# Autodesk Inventor assembly: ORBD Assembly
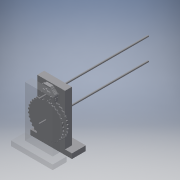
[picture p0: Inventor's stored thumbnail of the model, 180x180]
Saved by Autodesk Inventor 2017 (Build 210142000, 142)
## iProperties
Created: 2018-03-04
Part Number: ORBD Assembly
Document SubType Name: Assembly
Designer: Russ
Author: Russ
## Documents named in this file (5)
- C:\Users\Russ\Desktop\3D Models\ORBD\ORBD Assembly.iam
- C:\Users\Russ\Desktop\3D Models\ORBD\Braille Wheel.ipt
- C:\Users\Russ\Desktop\3D Models\ORBD\Middle Gear.ipt
- C:\Users\Russ\Desktop\3D Models\ORBD\Frame.ipt
- C:\Users\Russ\Desktop\3D Models\ORBD\Axle.ipt
## Components (8 placed, 4 different names)
1. Braille Wheel:1 — Mate:1, Mate:5, Mate:6, Rotation:1, Mate:9, Angle:1
2. Middle Gear:1 — Mate:1, Mate:3, Mate:4, Rotation:1
3. Frame:1 — Mate:3, Mate:4, Mate:5, Mate:6, Flush:2, Flush:3, Mate:7, Mate:8, Angle:1, Angle:2, Flush:4, Flush:5
4. Axle:1 — Flush:3, Mate:8, Mate:12
5. Axle:2 — Flush:2, Mate:7, Mate:10
6. Braille Wheel:2 — Mate:9, Mate:10, Mate:11, Rotation:2, Angle:2
7. Middle Gear:2 — Mate:11, Mate:12, Rotation:2, Mate:13
8. Frame:2 — Mate:13, Flush:4, Flush:5
## Relationships (20: Mate 12, Flush 4, RelateRotation 2, Angle 2)
- Mate:1: Braille Wheel:1 ↔ Middle Gear:1
- Mate:3: Middle Gear:1 ↔ Frame:1
- Mate:4: Middle Gear:1 ↔ Frame:1
- Mate:5: Braille Wheel:1 ↔ Frame:1
- Mate:6: Braille Wheel:1 ↔ Frame:1
- Flush:2: Frame:1 ↔ Axle:2
- Flush:3: Frame:1 ↔ Axle:1
- Mate:7: Frame:1 ↔ Axle:2
- Mate:8: Frame:1 ↔ Axle:1
- Rotation:1 [RelateRotation] (4 ul): Braille Wheel:1 ↔ Middle Gear:1
- Mate:9: Braille Wheel:1 ↔ Braille Wheel:2
- Mate:10: Axle:2 ↔ Braille Wheel:2
- Mate:11: Braille Wheel:2 ↔ Middle Gear:2
- Mate:12: Axle:1 ↔ Middle Gear:2
- Rotation:2 [RelateRotation] (4 ul): Braille Wheel:2 ↔ Middle Gear:2
- Angle:1 (0 deg): Braille Wheel:1 ↔ Frame:1
- Angle:2 (0 deg): Frame:1 ↔ Braille Wheel:2
- Mate:13: Middle Gear:2 ↔ Frame:2
- Flush:4: Frame:1 ↔ Frame:2
- Flush:5: Frame:1 ↔ Frame:2
